# Autodesk Inventor assembly: Glyptodon
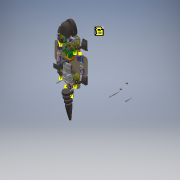
[picture p0: Inventor's stored thumbnail of the model, 180x180]
Saved by Autodesk Inventor 2018 (Build 220112000, 112)
## iProperties
Created: 2018-10-19
Part Number: Glyptodon
Document SubType Name: Assembly
Designer: reide
Author: reide
## Documents named in this file (73)
- C:\Users\reide\OneDrive\Documents\Inventor\TSA\2019\Animatronics\Glyptodon\Glyptodon Work\Glyptodon.iam
- C:\Users\reide\OneDrive\Documents\Inventor\TSA\2019\Animatronics\Glyptodon\Glyptodon Work\Frame.ipt
- C:\Users\reide\OneDrive\Documents\Inventor\TSA\2019\Animatronics\Glyptodon\Glyptodon Work\Syringe Mounts\SyringeBaseSlotters.ipt
- C:\Users\reide\OneDrive\Documents\Inventor\TSA\2019\Animatronics\Glyptodon\Glyptodon Work\Syringe Mounts\SyringeServoBaseClamp.ipt
- C:\Users\reide\OneDrive\Documents\Inventor\TSA\2019\Animatronics\Glyptodon\Glyptodon Work\Syringe Mounts\SyringeServoBaseClamp_MIR.ipt
- C:\Users\reide\OneDrive\Documents\Inventor\TSA\2019\Animatronics\Glyptodon\Glyptodon Work\Syringe Mounts\SyringeMotorBase.ipt
- C:\Users\reide\OneDrive\Documents\Inventor\TSA\2019\Animatronics\Glyptodon\Glyptodon Work\Syringe Mounts\SyringeMotorBase_MIR.ipt
- C:\Users\reide\OneDrive\Documents\Inventor\TSA\2019\Animatronics\Glyptodon\Mock Parts\servo (2).ipt
- C:\Users\reide\OneDrive\Documents\Inventor\TSA\2019\Animatronics\Glyptodon\Glyptodon Work\Syringe Mounts\BaseSyringeRackWall.ipt
- C:\Users\reide\OneDrive\Documents\Inventor\TSA\2019\Animatronics\Glyptodon\Glyptodon Work\Syringe Mounts\SyringeAttachment.ipt
- C:\Users\reide\OneDrive\Documents\Inventor\TSA\2019\Animatronics\Glyptodon\Glyptodon Work\Syringe3mL\SyringeBody.ipt
- C:\Users\reide\OneDrive\Documents\Inventor\TSA\2019\Animatronics\Glyptodon\Glyptodon Work\Syringe3mL\SyringEnd.ipt
- C:\Users\reide\OneDrive\Documents\Inventor\TSA\2019\Animatronics\Glyptodon\Glyptodon Work\Arms\ArmTruss.iam
- C:\Users\reide\OneDrive\Documents\Inventor\TSA\2019\Animatronics\Glyptodon\Glyptodon Work\Arms\GuideArmConnector - Copy.ipt
- C:\Users\reide\OneDrive\Documents\Inventor\TSA\2019\Animatronics\Glyptodon\Glyptodon Work\Arms\Roller_Wheel.ipt
- C:\Users\reide\OneDrive\Documents\Inventor\TSA\2019\Animatronics\Glyptodon\Glyptodon Work\Arms\Supporter.ipt
- C:\Users\reide\OneDrive\Documents\Inventor\TSA\2019\Animatronics\Glyptodon\Glyptodon Work\Arms\Rack.ipt
- C:\Users\reide\OneDrive\Documents\Inventor\TSA\2019\Animatronics\Glyptodon\Glyptodon Work\Arms\ArmTruss_MIR.iam
- C:\Users\reide\OneDrive\Documents\Inventor\TSA\2019\Animatronics\Glyptodon\Glyptodon Work\Front Wheel Drive\correct_wheel.ipt
- C:\Users\reide\OneDrive\Documents\Inventor\TSA\2019\Animatronics\Glyptodon\Glyptodon Work\Front Wheel Drive\wheel gear.ipt
- C:\Users\reide\OneDrive\Documents\Inventor\TSA\2019\Animatronics\Glyptodon\Glyptodon Work\Front Wheel Drive\wheelframe.ipt
- C:\Users\reide\OneDrive\Documents\Inventor\TSA\2019\Animatronics\Glyptodon\Glyptodon Work\Front Wheel Drive\wheelframe2NEW.ipt
- C:\Users\reide\OneDrive\Documents\Inventor\TSA\2019\Animatronics\Glyptodon\Glyptodon Work\Front Wheel Drive\WheelRing.ipt
- C:\Users\reide\OneDrive\Documents\Inventor\TSA\2019\Animatronics\Glyptodon\Glyptodon Work\Front Wheel Drive\smallergear.ipt
- C:\Users\reide\OneDrive\Documents\Inventor\TSA\2019\Animatronics\Glyptodon\Glyptodon Work\Front Wheel Drive\steer_servo_mount1.ipt
- C:\Users\reide\OneDrive\Documents\Inventor\TSA\2019\Animatronics\Glyptodon\Glyptodon Work\Front Wheel Drive\steer_servo_mount2.ipt
- C:\Users\reide\OneDrive\Documents\Inventor\TSA\2019\Animatronics\Glyptodon\Glyptodon Work\Front Wheel Drive\SteerServoClamp.ipt
- C:\Users\reide\OneDrive\Documents\Inventor\TSA\2019\Animatronics\Glyptodon\Glyptodon Work\Syringe Mounts\Pinion final.ipt
- C:\Users\reide\OneDrive\Documents\Inventor\TSA\2019\Animatronics\Glyptodon\Glyptodon Work\Front Wheel Drive\SwerveDriveClasp.ipt
- C:\Users\reide\OneDrive\Documents\Inventor\TSA\2019\Animatronics\Glyptodon\Glyptodon Work\Back Wheel Drive\BackWheelMount.ipt
- C:\Users\reide\OneDrive\Documents\Inventor\TSA\2019\Animatronics\Glyptodon\Glyptodon Work\Back Wheel Drive\BackWheelServoClasp.ipt
- C:\Users\reide\OneDrive\Documents\Inventor\TSA\2019\Animatronics\Glyptodon\Glyptodon Work\Table\TablePt1.ipt
- C:\Users\reide\OneDrive\Documents\Inventor\TSA\2019\Animatronics\Glyptodon\Glyptodon Work\Table\TablePt2.ipt
- C:\Users\reide\OneDrive\Documents\Inventor\TSA\2019\Animatronics\Glyptodon\Glyptodon Work\Tail\Tail_Mount.ipt
- C:\Users\reide\OneDrive\Documents\Inventor\TSA\2019\Animatronics\Glyptodon\Glyptodon Work\Tail\SyringeAttachmentTall.ipt
- C:\Users\reide\OneDrive\Documents\Inventor\TSA\2019\Animatronics\Glyptodon\Glyptodon Work\Tail\Tail3.ipt
- C:\Users\reide\OneDrive\Documents\Inventor\TSA\2019\Animatronics\Glyptodon\Glyptodon Work\Tail\SyringeTailLeverAttachment.ipt
- C:\Users\reide\OneDrive\Documents\Inventor\TSA\2019\Animatronics\Glyptodon\Glyptodon Work\Tail\SyringeBarTail.ipt
- C:\Users\reide\OneDrive\Documents\Inventor\TSA\2019\Animatronics\Glyptodon\Glyptodon Work\Syringe Mounts\HeadOpenRack.ipt
- C:\Users\reide\OneDrive\Documents\Inventor\TSA\2019\Animatronics\Glyptodon\Glyptodon Work\Table\SyringeServoClamp.ipt
- C:\Users\reide\OneDrive\Documents\Inventor\TSA\2019\Animatronics\Glyptodon\Glyptodon Work\Tail\SyringeTailLeverAttachment_MIR.ipt
- C:\Users\reide\OneDrive\Documents\Inventor\TSA\2019\Animatronics\Glyptodon\Glyptodon Work\Head\SyringeHeadLeverAttachment.ipt
- C:\Users\reide\OneDrive\Documents\Inventor\TSA\2019\Animatronics\Glyptodon\Glyptodon Work\Head\LeverArm.ipt
- C:\Users\reide\OneDrive\Documents\Inventor\TSA\2019\Animatronics\Glyptodon\Glyptodon Work\Head\HeadLever.ipt
- C:\Users\reide\OneDrive\Documents\Inventor\TSA\2019\Animatronics\Glyptodon\Glyptodon Work\Head\HeadLeverAssemblyAttacher.ipt
- C:\Users\reide\OneDrive\Documents\Inventor\TSA\2019\Animatronics\Glyptodon\Glyptodon Work\Arms\ArmClamp1.ipt
- C:\Users\reide\OneDrive\Documents\Inventor\TSA\2019\Animatronics\Glyptodon\Glyptodon Work\Arms\ArmClamp2.ipt
- C:\Users\reide\OneDrive\Documents\Inventor\TSA\2019\Animatronics\Glyptodon\Glyptodon Work\Arms\Foot.ipt
- C:\Users\reide\OneDrive\Documents\Inventor\TSA\2019\Animatronics\Glyptodon\Glyptodon Work\Arms\ArmClamp2_MIR.ipt
- C:\Users\reide\OneDrive\Documents\Inventor\TSA\2019\Animatronics\Glyptodon\Glyptodon Work\Arms\Foot_MIR.ipt
- C:\Users\reide\OneDrive\Documents\Inventor\TSA\2019\Animatronics\Glyptodon\Glyptodon Work\Arms\BackFoot.ipt
- C:\Users\reide\OneDrive\Documents\Inventor\TSA\2019\Animatronics\Glyptodon\Glyptodon Work\Arms\BackFoot_MIR.ipt
- C:\Users\reide\OneDrive\Documents\Inventor\TSA\2019\Animatronics\Glyptodon\Glyptodon Work\Arms\FootRoller.ipt
- C:\Users\reide\OneDrive\Documents\Inventor\TSA\2019\Animatronics\Glyptodon\Glyptodon Work\Button\ButtonMount.ipt
- C:\Users\reide\OneDrive\Documents\Inventor\TSA\2019\Animatronics\Glyptodon\Glyptodon Work\Button\ButtonMount2.ipt
- C:\Users\reide\OneDrive\Documents\Inventor\TSA\2019\Animatronics\Glyptodon\Glyptodon Work\Head\HeadBottom1.ipt
- C:\Users\reide\OneDrive\Documents\Inventor\TSA\2019\Animatronics\Glyptodon\Glyptodon Work\Head\Head1.ipt
- C:\Users\reide\OneDrive\Documents\Inventor\TSA\2019\Animatronics\Glyptodon\Glyptodon Work\Head\HeadChin.ipt
- C:\Users\reide\OneDrive\Documents\Inventor\TSA\2019\Animatronics\Glyptodon\Glyptodon Work\Head\Head2.ipt
- C:\Users\reide\OneDrive\Documents\Inventor\TSA\2019\Animatronics\Glyptodon\Glyptodon Work\Head\HeadFace.ipt
- C:\Users\reide\OneDrive\Documents\Inventor\TSA\2019\Animatronics\Glyptodon\Glyptodon Work\Head\HeadFlexHinge.ipt
- C:\Users\reide\OneDrive\Documents\Inventor\TSA\2019\Animatronics\Glyptodon\Glyptodon Work\Tail\Tail4.ipt
- C:\Users\reide\OneDrive\Documents\Inventor\TSA\2019\Animatronics\Glyptodon\Glyptodon Work\Tail\Tail5.ipt
- C:\Users\reide\OneDrive\Documents\Inventor\TSA\2019\Animatronics\Glyptodon\Glyptodon Work\Tail\Tail6.ipt
- C:\Users\reide\OneDrive\Documents\Inventor\TSA\2019\Animatronics\Glyptodon\Glyptodon Work\Arms\GuideArm.ipt
- C:\Users\reide\OneDrive\Documents\Inventor\TSA\2019\Animatronics\Glyptodon\Glyptodon Work\Arms\GuideArmConnectorLimitSwitch - Copy.ipt
- C:\Users\reide\OneDrive\Documents\3d Printing\Printrbot Metal\TSA\2019\Glyptodon\Arms\SensorMountV2.ipt
- C:\Users\reide\OneDrive\Documents\Inventor\TSA\2019\Animatronics\Glyptodon\Glyptodon Work\Button and Mounting\Imported Components\Backwheel\Backwheel.ipt
- C:\Users\reide\OneDrive\Documents\Inventor\TSA\2019\Animatronics\Glyptodon\Glyptodon Work\Button and Mounting\Imported Components\bump mount drill boi\bump mount drill boi.ipt
- C:\Users\reide\OneDrive\Documents\Inventor\TSA\2019\Animatronics\Glyptodon\Glyptodon Work\Button and Mounting\Imported Components\bump mount\bump mount.ipt
- C:\Users\reide\OneDrive\Documents\Inventor\TSA\2019\Animatronics\Glyptodon\Glyptodon Work\Button and Mounting\Imported Components\food_nug_pegs\food_nug_pegs.ipt
- C:\Users\reide\OneDrive\Documents\Inventor\TSA\2019\Animatronics\Glyptodon\Glyptodon Work\Button and Mounting\Imported Components\food_nug_pegs^-1\food_nug_pegs^-1.ipt
- C:\Users\reide\OneDrive\Documents\Inventor\TSA\2019\Animatronics\Glyptodon\Glyptodon Work\Button and Mounting\Imported Components\shell peg boi\shell peg boi.ipt
## Components (151 placed, 72 different names)
1. Frame:1 — Mate:8, Mate:9, Mate:10, Mate:11, Mate:12, Mate:13, Mate:14, Mate:15, Mate:17, Mate:20, Mate:23, Mate:24, Mate:25, Mate:28, Mate:31, Mate:38, Mate:39, Mate:40, Mate:41, Mate:42, Mate:43, Mate:44, Mate:45, Mate:72, Mate:73, Mate:106, Mate:107, Mate:108, Mate:109, Mate:110, Mate:113, Mate:114, Mate:115, Mate:118, Mate:119, Mate:139, Mate:140, Flush:56, Mate:147, Mate:148, Mate:149, Mate:150, Mate:151, Mate:152, Mate:153, Mate:155, Mate:157, Flush:57, Mate:161, Mate:168, Mate:176, Mate:180, Mate:181, Mate:182, Mate:183, Mate:184, Mate:204, Mate:205, Mate:206, Mate:207, Mate:208, Mate:209, Mate:210, Angle:11, Angle:12, Mate:242, Mate:245, Mate:310, Mate:311, Mate:312, Mate:360, Mate:361, Mate:362, Mate:363, Mate:364, Mate:366, Mate:376, Mate:377, Mate:383, Mate:384, Mate:385, Mate:401, Mate:402, Mate:403, Mate:406, Mate:407, Mate:408, Mate:410, Mate:411, Mate:412, Mate:416, Mate:418, Mate:420
2. SyringeBaseSlotters:1 — Mate:13, Mate:14, Mate:15, Mate:26, Mate:27, Mate:29, Mate:30, Flush:9
3. SyringeServoBaseClamp:1 — Mate:4, Flush:2, Flush:3
4. SyringeServoBaseClamp_MIR:1 — Mate:7, Flush:6, Flush:7
5. SyringeMotorBase:1 — Mate:2, Mate:3, Flush:1, Mate:4, Flush:2, Flush:3, Flush:4, Mate:11, Mate:12
6. SyringeMotorBase_MIR:1 — Flush:4, Mate:5, Mate:6, Flush:5, Mate:7, Flush:6, Flush:7, Mate:8, Mate:9, Mate:10, Flush:8, Mate:243
7. servo (2):1 — Mate:2, Mate:3, Flush:1, Mate:144, Mate:145
8. servo (2):2 — Mate:5, Mate:6, Flush:5, Mate:142, Mate:143
9. BaseSyringeRackWall:1 — Mate:17, Flush:8
10. SyringeAttachment:1 — Mate:25, Mate:26, Mate:27
11. BaseSyringeRackWall:2 — Mate:20, Mate:23, Mate:24, Mate:246
12. SyringeAttachment:2 — Mate:28, Mate:29, Mate:30, Mate:32, Mate:46, Flush:11
13. SyringeBaseSlotters:2 — Mate:31, Mate:32, Flush:9
14. SyringeBaseSlotters:3 — Mate:38, Mate:42, Mate:43
15. SyringeAttachment:3 — Mate:45
16. SyringeAttachment:4 — Mate:44, Mate:52, Flush:12
17. SyringeBaseSlotters:4 — Mate:39, Mate:40, Mate:41
18. SyringeBody:1 — Mate:46, Flush:11, Mate:49, Angle:11
19. SyringEnd:1 — Mate:49, Mate:244
20. SyringeBody:2 — Mate:52, Flush:12, Angle:12
21. SyringEnd:2 — Mate:247
22. ArmTruss:1 [sub-assembly] — Mate:62, Flush:21, Mate:63, Mate:300, Mate:301, Mate:302, Mate:404, Mate:405
23. Roller_Wheel:1 — Mate:68, Mate:69
24. Supporter:1 — Angle:1, Flush:24, Mate:73, Angle:7, Mate:404
25. Rack:1 — Flush:23, Mate:106, Mate:107
26. servo (2):3 — Mate:62, Flush:21, Mate:63, Angle:1, Mate:70, Mate:71
27. Supporter:2 — Angle:2, Flush:23, Mate:72, Mate:395
28. ArmTruss_MIR:1 [sub-assembly] — Angle:2, Mate:66, Flush:22, Mate:67, Mate:291, Mate:292, Mate:293, Mate:396
29. servo (2):4 — Mate:66, Flush:22, Mate:67, Mate:68, Mate:69, Mate:395
30. Roller_Wheel:2 — Mate:70, Mate:71
31. Rack:2 — Flush:24, Mate:108, Mate:109, Mate:190
32. ArmTruss:2 [sub-assembly] — Mate:268, Mate:269, Mate:270, Mate:386
33. Supporter:3 — Mate:115, Mate:387
34. servo (2):5 — Mate:387
35. Roller_Wheel:3
36. Rack:3 — Mate:118, Mate:119
37. Roller_Wheel:4
38. Rack:4 — Mate:113, Mate:114
39. Supporter:4 — Mate:110, Mate:414
40. ArmTruss_MIR:2 [sub-assembly] — Mate:279, Mate:280, Mate:281, Mate:415
41. servo (2):6 — Mate:414
42. correct_wheel:1
43. wheel gear:1
44. wheelframe:1 — Mate:137, Flush:70
45. wheelframe2NEW:1 — Mate:140
46. servo (2):7 — Flush:70
47. WheelRing:1 — Mate:137, Mate:139
48. smallergear:1
49. steer_servo_mount1:1 — Mate:167, Flush:72
50. steer_servo_mount2:1
51. SteerServoClamp:1
52. servo (2):8
53. steer_servo_mount2:2
54. Pinion final:1 — Mate:142, Mate:143
55. Pinion final:2 — Mate:144, Mate:145
56. SwerveDriveClasp:1 — Flush:56, Mate:147
57. SwerveDriveClasp:2 — Mate:148, Mate:153
58. SwerveDriveClasp:3 — Mate:149, Mate:152
59. SwerveDriveClasp:4 — Mate:150, Mate:151
60. BackWheelMount:1 — Mate:155, Mate:157, Flush:57, Mate:375
61. BackWheelServoClasp:1 — Mate:158, Mate:159, Mate:160, Mate:161
62. servo (2):9 — Mate:158, Mate:159, Mate:160
63. TablePt1:1 — Flush:58, Flush:59, Mate:164, Mate:168, Mate:223, Mate:224, Mate:225, Mate:226, Mate:227, Mate:228
64. TablePt2:1 — Flush:58, Flush:59, Mate:164, Mate:167, Mate:233, Mate:234, Mate:235, Mate:236, Mate:237, Mate:241, Flush:68, Flush:69
65. SyringeBaseSlotters:5 — Flush:64, Mate:176, Mate:186, Mate:187, Mate:188, Mate:190, Mate:193, Angle:8
66. SyringeBaseSlotters:6 — Flush:64, Angle:7, Mate:185, Mate:191, Mate:192
67. SyringeBody:3 — Mate:189, Mate:193, Angle:8
68. SyringEnd:3 — Mate:254, Mate:255
69. Tail_Mount:1 — Mate:180, Mate:181, Mate:182, Mate:192, Mate:194, Mate:195
70. SyringeAttachmentTall:1 — Mate:184, Mate:187, Mate:188, Mate:189, Mate:191
71. SyringeAttachmentTall:2 — Mate:183, Mate:185, Mate:186
72. Tail3:1 — Mate:194, Mate:195, Mate:213, Mate:219, Mate:351, Mate:352
73. SyringeBaseSlotters:7 — Mate:204, Mate:206
74. SyringeBaseSlotters:8 — Mate:205, Mate:207, Mate:208
75. SyringeBody:4
76. SyringEnd:4 — Mate:250, Mate:251
77. SyringeAttachmentTall:3 — Mate:210
78. SyringeAttachmentTall:4 — Mate:209
79. SyringeBarTail:2 — Mate:213, Mate:252, Mate:253
80. SyringeBarTail:3 — Mate:219, Mate:248, Mate:249
81. SyringeAttachment:5 — Mate:223, Mate:224, Mate:225, Mate:229
82. SyringeAttachment:6 — Mate:226, Mate:227, Mate:228
83. SyringEnd:5 — Mate:230, Mate:238
84. SyringeBody:5 — Mate:229, Mate:230
85. servo (2):10 — Mate:233, Mate:234, Mate:235
86. Pinion final:3 — Mate:239, Mate:240, Flush:67
87. HeadOpenRack:1 — Mate:236, Mate:237, Mate:238
88. Pinion final:4 — Mate:239, Mate:240, Flush:67
89. SyringeServoClamp:1 — Mate:241, Flush:68, Flush:69
90. HeadOpenRack:2 — Mate:242, Mate:243, Mate:244
91. HeadOpenRack:3 — Mate:245, Mate:246, Mate:247
92. SyringeTailLeverAttachment:3 — Mate:248, Mate:249, Mate:250, Mate:251
93. SyringeTailLeverAttachment_MIR:1 — Mate:252, Mate:253, Mate:254, Mate:255
94. LeverArm:2 — Mate:330, Mate:331, Mate:334, Mate:336
95. HeadLever:2 — Mate:314, Mate:315, Mate:316, Mate:318, Mate:330, Mate:331, Mate:332, Mate:333, Mate:341
96. HeadLeverAssemblyAttacher:3 — Mate:313, Mate:314, Mate:315, Angle:13
97. ArmClamp2_MIR:2 — Mate:268, Mate:269, Mate:270, Mate:271, Mate:272, Mate:273
98. ArmClamp1:2 — Mate:271, Mate:272, Mate:273, Mate:274, Mate:275, Mate:278
99. Foot_MIR:2 — Mate:274, Mate:275, Mate:278, Mate:306, Mate:307
100. BackFoot:1 — Mate:303, Mate:304, Mate:305
101. Foot:4 — Mate:285, Mate:286, Mate:287, Flush:71
102. ArmClamp2:3 — Mate:279, Mate:280, Mate:281, Mate:282, Mate:283, Mate:284
103. ArmClamp1:3 — Mate:282, Mate:283, Mate:284, Mate:285, Mate:286, Mate:287
104. ArmClamp2:4 — Mate:292, Mate:293
105. ArmClamp1:4 — Mate:291, Mate:294, Mate:295, Mate:296
106. BackFoot_MIR:2 — Mate:294, Mate:295, Mate:296
107. ArmClamp2_MIR:3 — Mate:300, Mate:301, Mate:302
108. ArmClamp1:5 — Mate:303, Mate:304, Mate:305
109. FootRoller:1 — Flush:71
110. FootRoller:2 — Mate:306, Mate:307
111. ButtonMount:1 — Flush:72, Mate:308, Mate:309
112. ButtonMount2:2 — Mate:308, Mate:309
113. HeadBottom1:2 — Mate:310, Mate:311, Mate:312, Flush:73, Angle:13, Mate:321, Mate:322, Mate:323, Mate:324, Mate:325, Mate:326
114. Head1:1 — Flush:73, Mate:313, Mate:317, Flush:75, Mate:343, Mate:344, Mate:345, Mate:346, Mate:357, Mate:358, Mate:359
115. HeadLeverAssemblyAttacher:4 — Mate:316, Mate:317, Mate:318
116. SyringeAttachment:7 — Mate:324, Mate:325, Flush:74, Mate:328, Angle:14
117. SyringeAttachment:8 — Mate:321, Mate:322, Mate:323, Flush:74
118. SyringEnd:6 — Mate:327, Mate:337, Mate:338
119. SyringeBody:7 — Mate:326, Mate:327, Mate:328, Angle:14
120. SyringeHeadLeverAttachment:2 — Mate:334, Mate:335, Mate:336, Mate:337, Mate:338
121. LeverArm:3 — Mate:332, Mate:333, Mate:335
122. HeadChin:1 — Flush:75
123. Head2:1 — Mate:341, Mate:343, Mate:346, Mate:349, Mate:350
124. HeadFace:1 — Mate:349, Mate:350
125. HeadFlexHinge:2 — Mate:344, Mate:345
126. Tail4:1 — Mate:351, Mate:352, Mate:353, Mate:354
127. Tail5:1 — Mate:353, Mate:354, Mate:355, Mate:356
128. Tail6:1 — Mate:355, Mate:356
129. HeadFlexHinge:3 — Mate:357, Mate:358, Mate:359
130. GuideArm:1 — Mate:365, Mate:367, Mate:415
131. GuideArmConnector - Copy:1 — Mate:363, Mate:364, Mate:365, Mate:366, Mate:367, Mate:417, Flush:84
132. GuideArmConnectorLimitSwitch - Copy:1 — Mate:360, Mate:361, Mate:362
133. SensorMountV2:1
134. Backwheel:2 — Mate:375, Mate:376
135. bump mount drill boi:1
136. bump mount:1
137. food_nug_pegs:1
138. food_nug_pegs^-1:1
139. shell peg boi:1 — Mate:377
140. GuideArm:3 — Mate:381, Flush:78, Mate:382, Flush:79, Mate:386
141. GuideArmConnector - Copy:8 — Flush:79
142. GuideArmConnectorLimitSwitch - Copy:3 — Mate:381, Flush:78, Mate:382, Mate:383, Mate:384, Mate:385
143. GuideArm:4 — Mate:396, Mate:409, Mate:413
144. GuideArm:5 — Mate:405
145. GuideArmConnector - Copy:10
146. GuideArmConnectorLimitSwitch - Copy:5 — Mate:401, Mate:402, Mate:403, Flush:85, Mate:419
147. GuideArmConnectorLimitSwitch - Copy:6 — Mate:410, Mate:411, Mate:412, Mate:413, Flush:86, Mate:421
148. GuideArmConnector - Copy:11 — Mate:406, Mate:407, Mate:408, Mate:409
149. shell peg boi:2 — Mate:416, Mate:417, Flush:84
150. shell peg boi:3 — Mate:420, Flush:86, Mate:421
151. shell peg boi:4 — Mate:418, Flush:85, Mate:419
## Relationships (371: Mate 307, Flush 53, Angle 11)
- Mate:2: SyringeMotorBase:1 ↔ servo (2):1
- Mate:3 (0.25 mm): SyringeMotorBase:1 ↔ servo (2):1
- Flush:1: SyringeMotorBase:1 ↔ servo (2):1
- Mate:4: SyringeServoBaseClamp:1 ↔ SyringeMotorBase:1
- Flush:2: SyringeServoBaseClamp:1 ↔ SyringeMotorBase:1
- Flush:3: SyringeServoBaseClamp:1 ↔ SyringeMotorBase:1
- Flush:4: SyringeMotorBase:1 ↔ SyringeMotorBase_MIR:1
- Mate:5: SyringeMotorBase_MIR:1 ↔ servo (2):2
- Mate:6 (0.25 mm): SyringeMotorBase_MIR:1 ↔ servo (2):2
- Flush:5: SyringeMotorBase_MIR:1 ↔ servo (2):2
- Mate:7: SyringeServoBaseClamp_MIR:1 ↔ SyringeMotorBase_MIR:1
- Flush:6: SyringeServoBaseClamp_MIR:1 ↔ SyringeMotorBase_MIR:1
- Flush:7: SyringeServoBaseClamp_MIR:1 ↔ SyringeMotorBase_MIR:1
- Mate:8: Frame:1 ↔ SyringeMotorBase_MIR:1
- Mate:9: Frame:1 ↔ SyringeMotorBase_MIR:1
- Mate:10: Frame:1 ↔ SyringeMotorBase_MIR:1
- Mate:11: Frame:1 ↔ SyringeMotorBase:1
- Mate:12: Frame:1 ↔ SyringeMotorBase:1
- Mate:13: Frame:1 ↔ SyringeBaseSlotters:1
- Mate:14: Frame:1 ↔ SyringeBaseSlotters:1
- Mate:15: Frame:1 ↔ SyringeBaseSlotters:1
- Mate:17: Frame:1 ↔ BaseSyringeRackWall:1
- Flush:8: SyringeMotorBase_MIR:1 ↔ BaseSyringeRackWall:1
- Mate:20: Frame:1 ↔ BaseSyringeRackWall:2
- Mate:23: Frame:1 ↔ BaseSyringeRackWall:2
- Mate:24: Frame:1 ↔ BaseSyringeRackWall:2
- Mate:25: Frame:1 ↔ SyringeAttachment:1
- Mate:26: SyringeBaseSlotters:1 ↔ SyringeAttachment:1
- Mate:27 (0.25 mm): SyringeBaseSlotters:1 ↔ SyringeAttachment:1
- Mate:28: Frame:1 ↔ SyringeAttachment:2
- Mate:29 (0.25 mm): SyringeBaseSlotters:1 ↔ SyringeAttachment:2
- Mate:30: SyringeBaseSlotters:1 ↔ SyringeAttachment:2
- Mate:31: Frame:1 ↔ SyringeBaseSlotters:2
- Mate:32: SyringeAttachment:2 ↔ SyringeBaseSlotters:2
- Flush:9: SyringeBaseSlotters:1 ↔ SyringeBaseSlotters:2
- [Mate]: SyringeBaseSlotters:3 ↔ SyringeAttachment:3
- [Mate] (0.25 mm): SyringeBaseSlotters:3 ↔ SyringeAttachment:3
- [Mate] (0.25 mm): SyringeBaseSlotters:3 ↔ SyringeAttachment:4
- [Mate]: SyringeBaseSlotters:3 ↔ SyringeAttachment:4
- [Mate]: SyringeAttachment:4 ↔ SyringeBaseSlotters:4
- [Flush]: SyringeBaseSlotters:3 ↔ SyringeBaseSlotters:4
- Mate:38: Frame:1 ↔ SyringeBaseSlotters:3
- Mate:39: Frame:1 ↔ SyringeBaseSlotters:4
- Mate:40: Frame:1 ↔ SyringeBaseSlotters:4
- Mate:41: Frame:1 ↔ SyringeBaseSlotters:4
- Mate:42: Frame:1 ↔ SyringeBaseSlotters:3
- Mate:43: Frame:1 ↔ SyringeBaseSlotters:3
- Mate:44: Frame:1 ↔ SyringeAttachment:4
- Mate:45: Frame:1 ↔ SyringeAttachment:3
- Mate:46: SyringeAttachment:2 ↔ SyringeBody:1
- Flush:11 (-10 mm): SyringeAttachment:2 ↔ SyringeBody:1
- Mate:49: SyringeBody:1 ↔ SyringEnd:1
- [Mate]: SyringeBody:2 ↔ SyringEnd:2
- Mate:52: SyringeAttachment:4 ↔ SyringeBody:2
- Flush:12 (-10 mm): SyringeAttachment:4 ↔ SyringeBody:2
- Mate:62: ArmTruss:1 ↔ servo (2):3
- Flush:21: ArmTruss:1 ↔ servo (2):3
- Mate:63 (0.5 mm): ArmTruss:1 ↔ servo (2):3
- Angle:1 (0 deg): Supporter:1 ↔ servo (2):3
- Angle:2 (0 deg): Supporter:2 ↔ ArmTruss_MIR:1
- Mate:66: ArmTruss_MIR:1 ↔ servo (2):4
- Flush:22: ArmTruss_MIR:1 ↔ servo (2):4
- Mate:67 (0.5 mm): ArmTruss_MIR:1 ↔ servo (2):4
- Mate:68: Roller_Wheel:1 ↔ servo (2):4
- Mate:69: Roller_Wheel:1 ↔ servo (2):4
- Mate:70: servo (2):3 ↔ Roller_Wheel:2
- Mate:71: servo (2):3 ↔ Roller_Wheel:2
- Flush:23: Rack:1 ↔ Supporter:2
- Flush:24: Supporter:1 ↔ Rack:2
- Mate:72: Frame:1 ↔ Supporter:2
- Mate:73: Frame:1 ↔ Supporter:1
- [Mate]: ArmTruss:2 ↔ servo (2):5
- [Flush]: ArmTruss:2 ↔ servo (2):5
- [Mate] (0.5 mm): ArmTruss:2 ↔ servo (2):5
- [Angle] (0 deg): Supporter:3 ↔ servo (2):5
- [Mate]: servo (2):5 ↔ Roller_Wheel:3
- [Mate]: servo (2):5 ↔ Roller_Wheel:3
- [Flush]: Supporter:3 ↔ Rack:3
- [Angle] (0 deg): Supporter:4 ↔ ArmTruss_MIR:2
- [Mate]: ArmTruss_MIR:2 ↔ servo (2):6
- [Flush]: ArmTruss_MIR:2 ↔ servo (2):6
- [Mate] (0.5 mm): ArmTruss_MIR:2 ↔ servo (2):6
- [Mate]: Roller_Wheel:4 ↔ servo (2):6
- [Mate]: Roller_Wheel:4 ↔ servo (2):6
- [Flush]: Rack:4 ↔ Supporter:4
- Mate:106: Frame:1 ↔ Rack:1
- Mate:107: Frame:1 ↔ Rack:1
- Mate:108: Frame:1 ↔ Rack:2
- Mate:109: Frame:1 ↔ Rack:2
- Mate:110: Frame:1 ↔ Supporter:4
- Mate:113: Frame:1 ↔ Rack:4
- Mate:114: Frame:1 ↔ Rack:4
- Mate:115: Frame:1 ↔ Supporter:3
- Mate:118: Frame:1 ↔ Rack:3
- Mate:119: Frame:1 ↔ Rack:3
- [Mate]: wheelframe:1 ↔ wheelframe2NEW:1
- [Flush]: wheelframe:1 ↔ wheelframe2NEW:1
- [Mate]: wheelframe:1 ↔ wheelframe2NEW:1
- [Mate]: wheelframe:1 ↔ wheelframe2NEW:1
- [Mate]: wheelframe:1 ↔ servo (2):7
- [Mate]: wheel gear:1 ↔ servo (2):7
- [Mate]: correct_wheel:1 ↔ wheelframe:1
- [Flush]: correct_wheel:1 ↔ wheel gear:1
- [Flush]: wheelframe:1 ↔ WheelRing:1
- [Flush]: steer_servo_mount1:1 ↔ steer_servo_mount2:1
- [Flush]: steer_servo_mount1:1 ↔ steer_servo_mount2:1
- [Flush]: steer_servo_mount1:1 ↔ steer_servo_mount2:1
- [Flush]: steer_servo_mount1:1 ↔ steer_servo_mount2:1
- [Mate]: steer_servo_mount1:1 ↔ steer_servo_mount2:1
- [Mate]: steer_servo_mount1:1 ↔ steer_servo_mount2:2
- [Flush]: steer_servo_mount1:1 ↔ steer_servo_mount2:2
- [Flush]: steer_servo_mount1:1 ↔ steer_servo_mount2:2
- [Mate]: steer_servo_mount1:1 ↔ servo (2):8
- [Mate]: steer_servo_mount1:1 ↔ servo (2):8
- [Mate] (0.5 mm): steer_servo_mount1:1 ↔ servo (2):8
- [Mate]: smallergear:1 ↔ servo (2):8
- [Mate]: smallergear:1 ↔ servo (2):8
- [Mate]: steer_servo_mount1:1 ↔ SteerServoClamp:1
- [Mate]: steer_servo_mount1:1 ↔ SteerServoClamp:1
- [Mate]: steer_servo_mount1:1 ↔ SteerServoClamp:1
- Mate:137: wheelframe:1 ↔ WheelRing:1
- Mate:139: Frame:1 ↔ WheelRing:1
- Mate:140: Frame:1 ↔ wheelframe2NEW:1
- Mate:142: servo (2):2 ↔ Pinion final:1
- Mate:143: servo (2):2 ↔ Pinion final:1
- Mate:144: servo (2):1 ↔ Pinion final:2
- Mate:145: servo (2):1 ↔ Pinion final:2
- Flush:56: Frame:1 ↔ SwerveDriveClasp:1
- Mate:147: Frame:1 ↔ SwerveDriveClasp:1
- Mate:148: Frame:1 ↔ SwerveDriveClasp:2
- Mate:149: Frame:1 ↔ SwerveDriveClasp:3
- Mate:150: Frame:1 ↔ SwerveDriveClasp:4
- Mate:151: Frame:1 ↔ SwerveDriveClasp:4
- Mate:152: Frame:1 ↔ SwerveDriveClasp:3
- Mate:153: Frame:1 ↔ SwerveDriveClasp:2
- Mate:155: Frame:1 ↔ BackWheelMount:1
- Mate:157 (11.35 mm): Frame:1 ↔ BackWheelMount:1
- Flush:57: Frame:1 ↔ BackWheelMount:1
- Mate:158: BackWheelServoClasp:1 ↔ servo (2):9
- Mate:159 (1 mm): BackWheelServoClasp:1 ↔ servo (2):9
- Mate:160 (0.25 mm): BackWheelServoClasp:1 ↔ servo (2):9
- Mate:161: Frame:1 ↔ BackWheelServoClasp:1
- Flush:58: TablePt1:1 ↔ TablePt2:1
- Flush:59: TablePt1:1 ↔ TablePt2:1
- Mate:164: TablePt1:1 ↔ TablePt2:1
- Mate:167 (10 mm): steer_servo_mount1:1 ↔ TablePt2:1
- Mate:168: Frame:1 ↔ TablePt1:1
- [Flush]: SyringeBaseSlotters:5 ↔ SyringeBaseSlotters:6
- [Mate]: SyringeBody:3 ↔ SyringEnd:3
- Flush:64: SyringeBaseSlotters:5 ↔ SyringeBaseSlotters:6
- Mate:176: Frame:1 ↔ SyringeBaseSlotters:5
- Angle:7 (0 deg): Supporter:1 ↔ SyringeBaseSlotters:6
- Mate:180: Frame:1 ↔ Tail_Mount:1
- Mate:181: Frame:1 ↔ Tail_Mount:1
- Mate:182: Frame:1 ↔ Tail_Mount:1
- Mate:183: Frame:1 ↔ SyringeAttachmentTall:2
- Mate:184: Frame:1 ↔ SyringeAttachmentTall:1
- Mate:185: SyringeBaseSlotters:6 ↔ SyringeAttachmentTall:2
- Mate:186 (0.25 mm): SyringeBaseSlotters:5 ↔ SyringeAttachmentTall:2
- Mate:187: SyringeBaseSlotters:5 ↔ SyringeAttachmentTall:1
- Mate:188 (0.25 mm): SyringeBaseSlotters:5 ↔ SyringeAttachmentTall:1
- Mate:189: SyringeBody:3 ↔ SyringeAttachmentTall:1
- Mate:190: Rack:2 ↔ SyringeBaseSlotters:5
- Mate:191: SyringeBaseSlotters:6 ↔ SyringeAttachmentTall:1
- Mate:192: SyringeBaseSlotters:6 ↔ Tail_Mount:1
- Mate:193: SyringeBaseSlotters:5 ↔ SyringeBody:3
- Angle:8 (0 deg): SyringeBaseSlotters:5 ↔ SyringeBody:3
- Mate:194: Tail_Mount:1 ↔ Tail3:1
- Mate:195: Tail_Mount:1 ↔ Tail3:1
- [Flush]: SyringeBaseSlotters:7 ↔ SyringeBaseSlotters:8
- [Mate]: SyringeBody:4 ↔ SyringEnd:4
- [Flush]: SyringeBaseSlotters:7 ↔ SyringeBaseSlotters:8
- [Mate]: SyringeBaseSlotters:8 ↔ SyringeAttachmentTall:4
- [Mate] (0.25 mm): SyringeBaseSlotters:7 ↔ SyringeAttachmentTall:4
- [Mate]: SyringeBaseSlotters:7 ↔ SyringeAttachmentTall:3
- [Mate] (0.25 mm): SyringeBaseSlotters:7 ↔ SyringeAttachmentTall:3
- [Mate]: SyringeBody:4 ↔ SyringeAttachmentTall:3
- [Mate]: SyringeBaseSlotters:8 ↔ SyringeAttachmentTall:3
- [Mate]: SyringeBaseSlotters:7 ↔ SyringeBody:4
- [Angle] (0 deg): SyringeBaseSlotters:7 ↔ SyringeBody:4
- Mate:204: Frame:1 ↔ SyringeBaseSlotters:7
- Mate:205: Frame:1 ↔ SyringeBaseSlotters:8
- Mate:206: Frame:1 ↔ SyringeBaseSlotters:7
- Mate:207: Frame:1 ↔ SyringeBaseSlotters:8
- Mate:208: Frame:1 ↔ SyringeBaseSlotters:8
- Mate:209: Frame:1 ↔ SyringeAttachmentTall:4
- Mate:210: Frame:1 ↔ SyringeAttachmentTall:3
- Mate:213: Tail3:1 ↔ SyringeBarTail:2
- Mate:219: Tail3:1 ↔ SyringeBarTail:3
- Angle:11 (0 deg): Frame:1 ↔ SyringeBody:1
- Angle:12 (0 deg): Frame:1 ↔ SyringeBody:2
- Mate:223: TablePt1:1 ↔ SyringeAttachment:5
- Mate:224: TablePt1:1 ↔ SyringeAttachment:5
- Mate:225 (0.25 mm): TablePt1:1 ↔ SyringeAttachment:5
- Mate:226: TablePt1:1 ↔ SyringeAttachment:6
- Mate:227 (0.25 mm): TablePt1:1 ↔ SyringeAttachment:6
- Mate:228: TablePt1:1 ↔ SyringeAttachment:6
- Mate:229: SyringeAttachment:5 ↔ SyringeBody:5
- Mate:230: SyringEnd:5 ↔ SyringeBody:5
- [Mate]: servo (2):10 ↔ Pinion final:3
- [Mate]: servo (2):10 ↔ Pinion final:3
- Mate:233: TablePt2:1 ↔ servo (2):10
- Mate:234 (0.25 mm): TablePt2:1 ↔ servo (2):10
- Mate:235 (0.25 mm): TablePt2:1 ↔ servo (2):10
- Mate:236: TablePt2:1 ↔ HeadOpenRack:1
- Mate:237 (0.25 mm): TablePt2:1 ↔ HeadOpenRack:1
- Mate:238: SyringEnd:5 ↔ HeadOpenRack:1
- Mate:239: Pinion final:3 ↔ Pinion final:4
- Mate:240: Pinion final:3 ↔ Pinion final:4
- Flush:67: Pinion final:3 ↔ Pinion final:4
- Mate:241: TablePt2:1 ↔ SyringeServoClamp:1
- Flush:68: TablePt2:1 ↔ SyringeServoClamp:1
- Flush:69: TablePt2:1 ↔ SyringeServoClamp:1
- Mate:242: Frame:1 ↔ HeadOpenRack:2
- Mate:243 (0.25 mm): SyringeMotorBase_MIR:1 ↔ HeadOpenRack:2
- Mate:244: SyringEnd:1 ↔ HeadOpenRack:2
- Mate:245: Frame:1 ↔ HeadOpenRack:3
- Mate:246 (0.25 mm): BaseSyringeRackWall:2 ↔ HeadOpenRack:3
- Mate:247: SyringEnd:2 ↔ HeadOpenRack:3
- Mate:248: SyringeBarTail:3 ↔ SyringeTailLeverAttachment:3
- Mate:249: SyringeBarTail:3 ↔ SyringeTailLeverAttachment:3
- Mate:250: SyringEnd:4 ↔ SyringeTailLeverAttachment:3
- Mate:251: SyringEnd:4 ↔ SyringeTailLeverAttachment:3
- Mate:252: SyringeBarTail:2 ↔ SyringeTailLeverAttachment_MIR:1
- Mate:253: SyringeBarTail:2 ↔ SyringeTailLeverAttachment_MIR:1
- Mate:254: SyringEnd:3 ↔ SyringeTailLeverAttachment_MIR:1
- Mate:255: SyringEnd:3 ↔ SyringeTailLeverAttachment_MIR:1
- Flush:70: wheelframe:1 ↔ servo (2):7
- Mate:268: ArmTruss:2 ↔ ArmClamp2_MIR:2
- Mate:269 (0.25 mm): ArmTruss:2 ↔ ArmClamp2_MIR:2
- Mate:270 (0.25 mm): ArmTruss:2 ↔ ArmClamp2_MIR:2
- Mate:271: ArmClamp2_MIR:2 ↔ ArmClamp1:2
- Mate:272: ArmClamp2_MIR:2 ↔ ArmClamp1:2
- Mate:273: ArmClamp2_MIR:2 ↔ ArmClamp1:2
- Mate:274 (0.25 mm): ArmClamp1:2 ↔ Foot_MIR:2
- Mate:275 (0.25 mm): ArmClamp1:2 ↔ Foot_MIR:2
- Mate:278: ArmClamp1:2 ↔ Foot_MIR:2
- Mate:279: ArmTruss_MIR:2 ↔ ArmClamp2:3
- Mate:280 (0.25 mm): ArmTruss_MIR:2 ↔ ArmClamp2:3
- Mate:281 (0.25 mm): ArmTruss_MIR:2 ↔ ArmClamp2:3
- Mate:282: ArmClamp2:3 ↔ ArmClamp1:3
- Mate:283: ArmClamp2:3 ↔ ArmClamp1:3
- Mate:284: ArmClamp2:3 ↔ ArmClamp1:3
- Mate:285 (0.25 mm): Foot:4 ↔ ArmClamp1:3
- Mate:286: Foot:4 ↔ ArmClamp1:3
- Mate:287: Foot:4 ↔ ArmClamp1:3
- [Mate]: ArmClamp2:4 ↔ ArmClamp1:4
- [Mate]: ArmClamp2:4 ↔ ArmClamp1:4
- [Mate]: ArmClamp2:4 ↔ ArmClamp1:4
- Mate:291: ArmTruss_MIR:1 ↔ ArmClamp1:4
- Mate:292 (0.25 mm): ArmTruss_MIR:1 ↔ ArmClamp2:4
- Mate:293 (0.25 mm): ArmTruss_MIR:1 ↔ ArmClamp2:4
- Mate:294 (0.25 mm): ArmClamp1:4 ↔ BackFoot_MIR:2
- Mate:295: ArmClamp1:4 ↔ BackFoot_MIR:2
- Mate:296: ArmClamp1:4 ↔ BackFoot_MIR:2
- [Mate]: ArmClamp2_MIR:3 ↔ ArmClamp1:5
- [Mate]: ArmClamp2_MIR:3 ↔ ArmClamp1:5
- [Mate]: ArmClamp2_MIR:3 ↔ ArmClamp1:5
- Mate:300: ArmTruss:1 ↔ ArmClamp2_MIR:3
- Mate:301 (0.25 mm): ArmTruss:1 ↔ ArmClamp2_MIR:3
- Mate:302 (0.25 mm): ArmTruss:1 ↔ ArmClamp2_MIR:3
- Mate:303 (0.25 mm): BackFoot:1 ↔ ArmClamp1:5
- Mate:304: BackFoot:1 ↔ ArmClamp1:5
- Mate:305: BackFoot:1 ↔ ArmClamp1:5
- Flush:71: Foot:4 ↔ FootRoller:1
- Mate:306 (0.25 mm): Foot_MIR:2 ↔ FootRoller:2
- Mate:307: Foot_MIR:2 ↔ FootRoller:2
- Flush:72: steer_servo_mount1:1 ↔ ButtonMount:1
- Mate:308 (0.5 mm): ButtonMount:1 ↔ ButtonMount2:2
- Mate:309 (0.5 mm): ButtonMount:1 ↔ ButtonMount2:2
- Mate:310: Frame:1 ↔ HeadBottom1:2
- Mate:311: Frame:1 ↔ HeadBottom1:2
- Mate:312: Frame:1 ↔ HeadBottom1:2
- Flush:73: HeadBottom1:2 ↔ Head1:1
- Mate:313: HeadLeverAssemblyAttacher:3 ↔ Head1:1
- Mate:314 (0.5 mm): HeadLever:2 ↔ HeadLeverAssemblyAttacher:3
- Mate:315: HeadLever:2 ↔ HeadLeverAssemblyAttacher:3
- Mate:316 (0.5 mm): HeadLever:2 ↔ HeadLeverAssemblyAttacher:4
- Mate:317: Head1:1 ↔ HeadLeverAssemblyAttacher:4
- Mate:318: HeadLever:2 ↔ HeadLeverAssemblyAttacher:4
- Angle:13 (0 deg): HeadLeverAssemblyAttacher:3 ↔ HeadBottom1:2
- Mate:321: HeadBottom1:2 ↔ SyringeAttachment:8
- Mate:322 (0.25 mm): HeadBottom1:2 ↔ SyringeAttachment:8
- Mate:323 (0.25 mm): HeadBottom1:2 ↔ SyringeAttachment:8
- Mate:324 (0.25 mm): HeadBottom1:2 ↔ SyringeAttachment:7
- Mate:325 (0.25 mm): HeadBottom1:2 ↔ SyringeAttachment:7
- Flush:74: SyringeAttachment:7 ↔ SyringeAttachment:8
- Mate:326: HeadBottom1:2 ↔ SyringeBody:7
- Mate:327: SyringEnd:6 ↔ SyringeBody:7
- Mate:328: SyringeAttachment:7 ↔ SyringeBody:7
- Angle:14 (0 deg): SyringeAttachment:7 ↔ SyringeBody:7
- Mate:330: LeverArm:2 ↔ HeadLever:2
- Mate:331 (0.25 mm): LeverArm:2 ↔ HeadLever:2
- Mate:332 (0.25 mm): HeadLever:2 ↔ LeverArm:3
- Mate:333: HeadLever:2 ↔ LeverArm:3
- Mate:334: LeverArm:2 ↔ SyringeHeadLeverAttachment:2
- Mate:335: SyringeHeadLeverAttachment:2 ↔ LeverArm:3
- Mate:336: LeverArm:2 ↔ SyringeHeadLeverAttachment:2
- Mate:337: SyringEnd:6 ↔ SyringeHeadLeverAttachment:2
- Mate:338: SyringEnd:6 ↔ SyringeHeadLeverAttachment:2
- Flush:75: Head1:1 ↔ HeadChin:1
- Mate:341: HeadLever:2 ↔ Head2:1
- Mate:343: Head1:1 ↔ Head2:1
- Mate:344: Head1:1 ↔ HeadFlexHinge:2
- Mate:345: Head1:1 ↔ HeadFlexHinge:2
- Mate:346: Head1:1 ↔ Head2:1
- Mate:349: Head2:1 ↔ HeadFace:1
- Mate:350: Head2:1 ↔ HeadFace:1
- Mate:351: Tail3:1 ↔ Tail4:1
- Mate:352: Tail3:1 ↔ Tail4:1
- Mate:353: Tail4:1 ↔ Tail5:1
- Mate:354: Tail4:1 ↔ Tail5:1
- Mate:355: Tail5:1 ↔ Tail6:1
- Mate:356: Tail5:1 ↔ Tail6:1
- Mate:357: Head1:1 ↔ HeadFlexHinge:3
- Mate:358: Head1:1 ↔ HeadFlexHinge:3
- Mate:359: Head1:1 ↔ HeadFlexHinge:3
- Mate:360: Frame:1 ↔ GuideArmConnectorLimitSwitch - Copy:1
- Mate:361: Frame:1 ↔ GuideArmConnectorLimitSwitch - Copy:1
- Mate:362: Frame:1 ↔ GuideArmConnectorLimitSwitch - Copy:1
- Mate:363: Frame:1 ↔ GuideArmConnector - Copy:1
- Mate:364: Frame:1 ↔ GuideArmConnector - Copy:1
- Mate:365: GuideArm:1 ↔ GuideArmConnector - Copy:1
- Mate:366: Frame:1 ↔ GuideArmConnector - Copy:1
- Mate:367: GuideArm:1 ↔ GuideArmConnector - Copy:1
- Mate:375: BackWheelMount:1 ↔ Backwheel:2
- Mate:376 (3.5 mm): Frame:1 ↔ Backwheel:2
- Mate:377: Frame:1 ↔ shell peg boi:1
- [Mate]: GuideArm:3 ↔ GuideArmConnector - Copy:8
- [Mate]: GuideArm:3 ↔ GuideArmConnector - Copy:8
- Mate:381: GuideArm:3 ↔ GuideArmConnectorLimitSwitch - Copy:3
- Flush:78: GuideArm:3 ↔ GuideArmConnectorLimitSwitch - Copy:3
- Mate:382: GuideArm:3 ↔ GuideArmConnectorLimitSwitch - Copy:3
- Flush:79: GuideArm:3 ↔ GuideArmConnector - Copy:8
- Mate:383: Frame:1 ↔ GuideArmConnectorLimitSwitch - Copy:3
- Mate:384: Frame:1 ↔ GuideArmConnectorLimitSwitch - Copy:3
- Mate:385: Frame:1 ↔ GuideArmConnectorLimitSwitch - Copy:3
- Mate:386 (0.25 mm): ArmTruss:2 ↔ GuideArm:3
- Mate:387: Supporter:3 ↔ servo (2):5
- Mate:395: Supporter:2 ↔ servo (2):4
- Mate:396 (0.25 mm): ArmTruss_MIR:1 ↔ GuideArm:4
- [Mate]: GuideArm:5 ↔ GuideArmConnector - Copy:10
- [Mate]: GuideArm:5 ↔ GuideArmConnector - Copy:10
- [Mate]: GuideArm:5 ↔ GuideArmConnectorLimitSwitch - Copy:5
- [Flush]: GuideArm:5 ↔ GuideArmConnectorLimitSwitch - Copy:5
- [Mate]: GuideArm:5 ↔ GuideArmConnectorLimitSwitch - Copy:5
- [Flush]: GuideArm:5 ↔ GuideArmConnector - Copy:10
- Mate:401: Frame:1 ↔ GuideArmConnectorLimitSwitch - Copy:5
- Mate:402: Frame:1 ↔ GuideArmConnectorLimitSwitch - Copy:5
- Mate:403: Frame:1 ↔ GuideArmConnectorLimitSwitch - Copy:5
- Mate:404: ArmTruss:1 ↔ Supporter:1
- Mate:405 (0.25 mm): ArmTruss:1 ↔ GuideArm:5
- Mate:406: Frame:1 ↔ GuideArmConnector - Copy:11
- Mate:407: Frame:1 ↔ GuideArmConnector - Copy:11
- Mate:408: Frame:1 ↔ GuideArmConnector - Copy:11
- Mate:409: GuideArm:4 ↔ GuideArmConnector - Copy:11
- Mate:410: Frame:1 ↔ GuideArmConnectorLimitSwitch - Copy:6
- Mate:411: Frame:1 ↔ GuideArmConnectorLimitSwitch - Copy:6
- Mate:412: Frame:1 ↔ GuideArmConnectorLimitSwitch - Copy:6
- Mate:413: GuideArm:4 ↔ GuideArmConnectorLimitSwitch - Copy:6
- Mate:414: Supporter:4 ↔ servo (2):6
- Mate:415 (0.25 mm): ArmTruss_MIR:2 ↔ GuideArm:1
- Mate:416: Frame:1 ↔ shell peg boi:2
- Mate:417: GuideArmConnector - Copy:1 ↔ shell peg boi:2
- Flush:84: GuideArmConnector - Copy:1 ↔ shell peg boi:2
- Mate:418: Frame:1 ↔ shell peg boi:4
- Flush:85: GuideArmConnectorLimitSwitch - Copy:5 ↔ shell peg boi:4
- Mate:419: GuideArmConnectorLimitSwitch - Copy:5 ↔ shell peg boi:4
- Mate:420: Frame:1 ↔ shell peg boi:3
- Flush:86: GuideArmConnectorLimitSwitch - Copy:6 ↔ shell peg boi:3
- Mate:421: GuideArmConnectorLimitSwitch - Copy:6 ↔ shell peg boi:3
## Named parameters: d44_d36 = 0 mm, d45_d37 = 0.25 mm, d46_d39 = 0.25 mm, d47_d40 = 0 mm, d48_d42 = 0 mm, d49_d43 = 0 mm, d64_d62 = 0 mm, d129_d90 = 0 deg, d130_d98 = 0 mm, d131_d99 = 0 mm, d132_d101 = 0 mm, d133_d86 = 0 mm, d134_d87 = 0 mm, d135_d88 = 0.5 mm, d147_d92 = 0 deg, d148_d93 = 0 mm, d149_d94 = 0 mm, d150_d95 = 0.5 mm, d151_d96 = 0 mm, d152_d97 = 0 mm, d153_d100 = 0 mm, d173_d12 = 0 mm, d174_d13 = 0 mm, d175_d14 = 0 mm, d176_d15 = 0 mm, d177_d16 = 0 mm, d179_d18 = 0 mm, d180_d19 = 0 mm, d181_d20 = 0 mm, d182_d21 = 0.5 mm, d183_d22 = 0 mm, d185_d24 = 0 mm, d189_d11 = 0 mm, d192_d7 = 0 mm, d193_d8 = 0 mm, d194_d9 = 0 mm, d195_d10 = 0 mm, d197_d1 = 0 mm, d198_d2 = 0 mm, d199_d3 = 0 mm, d200_d4 = 0 mm, d247_d49_d43 = 0 mm, d248_d64_d62 = 0 mm, d277_d273 = 0 mm, d278_d274 = 0 deg, d279_d247_d49_d43 = 0 mm, d280_d248_d64_d62 = 0 mm, d281_d253 = 0 mm, d282_d265 = 0 mm, d283_d266 = 0.25 mm, d284_d267 = 0 mm, d285_d268 = 0.25 mm, d286_d269 = 0 mm, d287_d271 = 0 mm, d323_d207 = 0 mm, d324_d208 = 0 mm, d416_d410 = 0 mm, d417_d411 = 0 mm, d418_d412 = 0 mm, d425_d389 = 0 mm, d426_d390 = 0 mm, d427_d391 = 0 mm, d552_d535 = 0 mm, d553_d537 = 0 mm, d574_d554 = 0 mm, d575_d555 = 0 mm, d576_d556 = 0 mm, d577_d557 = 0 mm, d578_d552_d535 = 0 mm, d579_d553_d537 = 0 mm
